# Autodesk Inventor assembly: narrow high rectangular -0.1
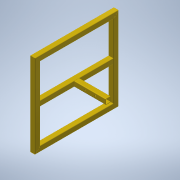
[picture p0: Inventor's stored thumbnail of the model, 180x180]
Saved by Autodesk Inventor 2021 (Build 250183000, 183)
## iProperties
Created: 2024-04-18
Part Number: narrow high rectangular -0.1
Document SubType Name: Assembly
Designer: Michal
Author: Michal
## Documents named in this file (4)
- C:\Users\Michal\Documents\GitHub\PNW_PhotoBoothFrame_3D\narrow high rectangular\narrow high rectangular -0.1.iam
- C:\Users\Michal\Documents\GitHub\PNW_PhotoBoothFrame_3D\narrow high rectangular\beam 25x25x2 1-3.ipt
- C:\Users\Michal\Documents\GitHub\PNW_PhotoBoothFrame_3D\narrow high rectangular\beam 25x25x2 1-2.ipt
- C:\Users\Michal\Documents\GitHub\PNW_PhotoBoothFrame_3D\narrow high rectangular\beam 25x25x2 1-1.ipt
## Components (6 placed, 3 different names)
1. beam 25x25x2 1-3:1 — Mate:1, Flush:1, Mate:2, Mate:5, Mate:6, Mate:8, Mate:10
2. beam 25x25x2 1-3:2 — Mate:1, Flush:1, Mate:2, Flush:2, Mate:3, Mate:7, Flush:4
3. beam 25x25x2 1-3:3 — Flush:2, Flush:3, Mate:3, Mate:4
4. beam 25x25x2 1-3:4 — Flush:3, Mate:4, Mate:5, Mate:6, Mate:9
5. beam 25x25x2 1-2:1 — Mate:7, Flush:4, Mate:11, Mate:12
6. beam 25x25x2 1-1:1 — Mate:12, Mate:13, Flush:5
## Relationships (18: Mate 13, Flush 5)
- Mate:1: beam 25x25x2 1-3:1 ↔ beam 25x25x2 1-3:2
- Flush:1: beam 25x25x2 1-3:1 ↔ beam 25x25x2 1-3:2
- Mate:2: beam 25x25x2 1-3:1 ↔ beam 25x25x2 1-3:2
- Flush:2: beam 25x25x2 1-3:2 ↔ beam 25x25x2 1-3:3
- Flush:3: beam 25x25x2 1-3:3 ↔ beam 25x25x2 1-3:4
- Mate:3: beam 25x25x2 1-3:2 ↔ beam 25x25x2 1-3:3
- Mate:4: beam 25x25x2 1-3:3 ↔ beam 25x25x2 1-3:4
- Mate:5: beam 25x25x2 1-3:1 ↔ beam 25x25x2 1-3:4
- Mate:6: beam 25x25x2 1-3:1 ↔ beam 25x25x2 1-3:4
- Mate:7: beam 25x25x2 1-3:2 ↔ beam 25x25x2 1-2:1
- Flush:4: beam 25x25x2 1-3:2 ↔ beam 25x25x2 1-2:1
- Mate:8: beam 25x25x2 1-3:1
- Mate:9: beam 25x25x2 1-3:4
- Mate:10: beam 25x25x2 1-3:1
- Mate:11: beam 25x25x2 1-2:1
- Mate:12: beam 25x25x2 1-2:1 ↔ beam 25x25x2 1-1:1
- Mate:13: beam 25x25x2 1-1:1
- Flush:5: beam 25x25x2 1-1:1
